# Autodesk Inventor assembly: Baugruppe1
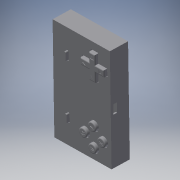
[picture p0: Inventor's stored thumbnail of the model, 180x180]
Saved by Autodesk Inventor 2019 (Build 230136000, 136)
## iProperties
Created: 2020-10-05
Part Number: Baugruppe1
Material: Generisch
Document SubType Name: Assembly
Designer: d_fel
Author: d_fel
## Documents named in this file (9)
- C:\Users\d_fel\Documents\HSR\Sem3.2\PmSwEng\Projekt\PC\PmSwEng\Baugruppe1.iam
- C:\Users\d_fel\Documents\HSR\Sem3.2\PmSwEng\Projekt\PC\PmSwEng\ButtonA_neu.ipt
- C:\Users\d_fel\Documents\HSR\Sem3.2\PmSwEng\Projekt\PC\PmSwEng\ButtonB_neu.ipt
- C:\Users\d_fel\Documents\HSR\Sem3.2\PmSwEng\Projekt\PC\PmSwEng\ButtonX_neu.ipt
- C:\Users\d_fel\Documents\HSR\Sem3.2\PmSwEng\Projekt\PC\PmSwEng\ButtonY_neu.ipt
- C:\Users\d_fel\Documents\HSR\Sem3.2\PmSwEng\Projekt\PC\PmSwEng\Front.ipt
- C:\Users\d_fel\Documents\HSR\Sem3.2\PmSwEng\Projekt\PC\PmSwEng\Kreuz.ipt
- C:\Users\d_fel\Documents\HSR\Sem3.2\PmSwEng\Projekt\PC\PmSwEng\startselectButton.ipt
- C:\Users\d_fel\Documents\HSR\Sem3.2\PmSwEng\Projekt\PC\PmSwEng\Bottom.ipt
## Components (9 placed, 8 different names)
1. ButtonA_neu:1 — Passend:15, Passend:16
2. ButtonB_neu:1 — Passend:1, Passend:17
3. ButtonX_neu:1 — Passend:13, Passend:14
4. ButtonY_neu:1 — Passend:3, Passend:18
5. Front:1 — Passend:1, Passend:3, Passend:5, Passend:6, Passend:7, Passend:8, Passend:9, Passend:10, Passend:11, Passend:12, Passend:13, Passend:14, Passend:15, Passend:16, Passend:17, Passend:18, Passend:19, Passend:20, Passend:21
6. Kreuz:1 — Passend:5, Passend:6, Passend:7, Passend:12
7. startselectButton:1 — Passend:9, Passend:11
8. startselectButton:2 — Passend:8, Passend:10
9. Bottom:1 — Passend:19, Passend:20, Passend:21
## Relationships (19: Mate 19)
- Passend:1 [Mate]: ButtonB_neu:1 ↔ Front:1
- Passend:3 [Mate]: ButtonY_neu:1 ↔ Front:1
- Passend:5 [Mate]: Front:1 ↔ Kreuz:1
- Passend:6 [Mate] (0.5 mm): Front:1 ↔ Kreuz:1
- Passend:7 [Mate] (0.5 mm): Front:1 ↔ Kreuz:1
- Passend:8 [Mate]: Front:1 ↔ startselectButton:2
- Passend:9 [Mate]: Front:1 ↔ startselectButton:1
- Passend:10 [Mate] (0.25 mm): Front:1 ↔ startselectButton:2
- Passend:11 [Mate] (0.25 mm): Front:1 ↔ startselectButton:1
- Passend:12 [Mate] (0.5 mm): Front:1 ↔ Kreuz:1
- Passend:13 [Mate]: ButtonX_neu:1 ↔ Front:1
- Passend:14 [Mate]: ButtonX_neu:1 ↔ Front:1
- Passend:15 [Mate]: ButtonA_neu:1 ↔ Front:1
- Passend:16 [Mate]: ButtonA_neu:1 ↔ Front:1
- Passend:17 [Mate]: ButtonB_neu:1 ↔ Front:1
- Passend:18 [Mate]: ButtonY_neu:1 ↔ Front:1
- Passend:19 [Mate]: Front:1 ↔ Bottom:1
- Passend:20 [Mate] (0.1 mm): Front:1 ↔ Bottom:1
- Passend:21 [Mate] (0.1 mm): Front:1 ↔ Bottom:1
